# Autodesk Inventor assembly: CL4-100
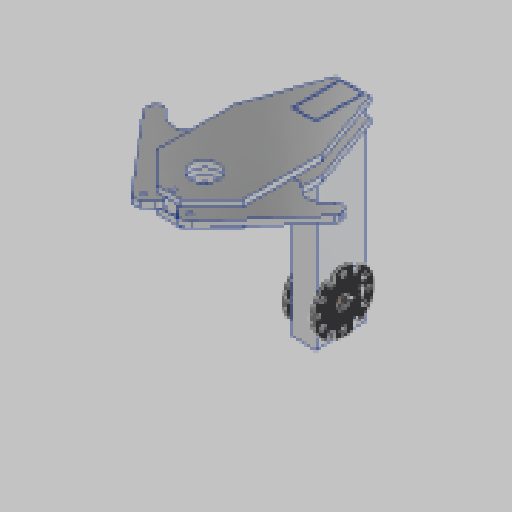
[picture p0: Inventor's stored thumbnail of the model, 512x512]
Saved by Autodesk Inventor 2023.5 (Build 275446000, 446)
## iProperties
Created: 2025-02-04
Part Number: CL4-100
Document SubType Name: Assembly
Designer: brand
Author: brand
## Documents named in this file (9)
- C:\Users\slick\OneDrive\Desktop\2025-ReefScape---CAD\Climber\CL4\CL4-100.iam
- C:\Users\slick\OneDrive\Desktop\2025-ReefScape---CAD\Climber\CL4\CL4-001.ipt
- C:\Users\slick\OneDrive\Desktop\2025-ReefScape---CAD\Climber\CL4\CL4-004.ipt
- C:\Users\slick\OneDrive\Desktop\2025-ReefScape---CAD\Field Items\Full Field\FE-2025\GE-25201.iam
- C:\Users\slick\OneDrive\Desktop\2025-ReefScape---CAD\Climber\CL4\02_Barb Assembly (1)\02_Barb Assembly (1).iam
- C:\Users\slick\OneDrive\Desktop\2025-ReefScape---CAD\Climber\CL4\CL4-005.ipt
- C:\Users\slick\OneDrive\Desktop\2025-ReefScape---CAD\Climber\CL4\CL4-006.ipt
- C:\Users\slick\OneDrive\Desktop\2025-ReefScape---CAD\COMMON PARTS\HUBS\WCP-1388.ipt
- C:\Users\slick\OneDrive\Desktop\2025-ReefScape---CAD\Climber\CL4\CL4-017.ipt
## Components (11 placed, 8 different names)
1. CL4-001:1 — Mate:7, Flush:6, Flush:7, Flush:8, Insert:2, Mate:14, Insert:3, Mate:15, Mate:16, Mate:17, Mate:20, Mate:21, Flush:10
2. CL4-005:1 — Flush:8, Flush:9, Mate:8, Mate:11, Mate:17
3. CL4-005:2 — Flush:9, Mate:8, Mate:9, Mate:10, Mate:12, Insert:1
4. CL4-004:1 — Mate:2, Mate:5, Mate:11, Mate:13, Mate:19
5. CL4-004:2 — Mate:2, Mate:5, Mate:9, Mate:10, Mate:12, Mate:13, Mate:18
6. GE-25201:1 [sub-assembly] — Mate:7
7. 02_Barb Assembly (1):1 [sub-assembly] — Flush:6, Flush:7
8. CL4-006:1 — Insert:1, Mate:18, Mate:19
9. WCP-1388:1 — Insert:2, Mate:14
10. WCP-1388:2 — Insert:3, Mate:15
11. CL4-017:1 — Mate:20, Mate:21, Flush:10
## Relationships (26: Mate 17, Flush 6, Insert 3)
- Mate:2: CL4-004:1 ↔ CL4-004:2
- Mate:5: CL4-004:1 ↔ CL4-004:2
- [Flush]: CL4-001:1 ↔ CL4-005:1
- Mate:7: CL4-001:1 ↔ GE-25201:1
- Flush:6: CL4-001:1 ↔ 02_Barb Assembly (1):1
- Flush:7: CL4-001:1 ↔ 02_Barb Assembly (1):1
- Flush:8: CL4-001:1 ↔ CL4-005:1
- Flush:9: CL4-005:1 ↔ CL4-005:2
- Mate:8: CL4-005:1 ↔ CL4-005:2
- Mate:9: CL4-005:2 ↔ CL4-004:2
- Mate:10: CL4-005:2 ↔ CL4-004:2
- Mate:11: CL4-005:1 ↔ CL4-004:1
- Mate:12: CL4-005:2 ↔ CL4-004:2
- Mate:13: CL4-004:1 ↔ CL4-004:2
- Insert:1: CL4-005:2 ↔ CL4-006:1
- Insert:2: CL4-001:1 ↔ WCP-1388:1
- Mate:14: CL4-001:1 ↔ WCP-1388:1
- Insert:3: CL4-001:1 ↔ WCP-1388:2
- Mate:15: CL4-001:1 ↔ WCP-1388:2
- Mate:16: CL4-001:1
- Mate:17: CL4-001:1 ↔ CL4-005:1
- Mate:18: CL4-004:2 ↔ CL4-006:1
- Mate:19: CL4-004:1 ↔ CL4-006:1
- Mate:20: CL4-001:1 ↔ CL4-017:1
- Mate:21: CL4-001:1 ↔ CL4-017:1
- Flush:10: CL4-001:1 ↔ CL4-017:1
